# Autodesk Inventor assembly: GEYK1.0-70-10-B-10K
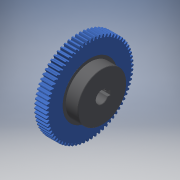
[picture p0: Inventor's stored thumbnail of the model, 180x180]
Saved by Autodesk Inventor 2019 (Build 230136000, 136)
## iProperties
Category: PARTsolutions
Company: MISUMI
Created: 2022-11-14
Part Number: GEYK1.0-70-10-B-10K
Catalog Web Link: www.cadenas.de
Description: GEY_-Plastic Bonded Spur Gears
Vendor: MISUMI
Document SubType Name: Assembly
Designer: psAdmin
Manufacturer: MISUMI
Mass: 49.0279 g
Surface Area: 167.17 cm^2
Volume: 49.0279 cm^3
Density: 1 g/cm^3
Title: GEYK1.0-70-10-B-10K
Author: Cadenas PARTsolutions
Comments: Plastic Bonded Spur Gears
PSOL_IDENT_0: {$CADENAS_DATA/23d-libs/misumi/metric/54_spur_gears/gey_asmtab.prj},217 {VTYP=3D},{STYP=ASSTAB},{NB=
PSOL_IDENT_1: GEYK1.0-70-10-B-10K},{LINA=GEYK1.0-70-10-B-10K},{NN=GEY_},{DATE=07.06.2021 01:25:59},{GEOMDATE=22.08
PSOL_IDENT_2: .2016 06:34:21},{VERSION=},{LINEID=10},{WBVAR=SHS,NT,PS,ALT1,ALT2,BS},{WBNUMERIC=NT,BS}  {NB=GEYK1.0
PSOL_IDENT_3: -70-10-B-10K},{LINA=GEYK1.0-70-10-B-10K},{KT=DUMMY},{PN=GEYK1.0-70-10-B-10K},{SHS=K},{SHSPN=K},{GEAK
PSOL_IDENT_4: BH=0},{MAT=MC Nylon},{MATC=S25C},{AC=Set Screw},{MOD=1.0},{NT=70},{NTA=30,32,34,35,36,38,40,42,45,48
PSOL_IDENT_5: ,50,52,56,60,70,75},{B=10},{TS=B},{TSA='B','B'},{PS=10K},{PSA= '10N','10N','10K','10K','11N','11N','
PSOL_IDENT_6: 12N','12N','13N','13N','14N','14N','15N','15N','16N','16N','17N','17N','18N','18N','19N','19N','20N'
PSOL_IDENT_7: ,'20N','21N','21N','22N','22N','23N','23N','24N','24N'},{PS1= '10','10','11','11','12','12','13','13'
PSOL_IDENT_8: ,'14','14','15','15','16','16','17','17','18','18','19','19','20','20','21','21','22','22','23','23'
PSOL_IDENT_9: ,'24','24','25','25','26','26','27','27','28','28'},{PS2= '10N','10N','10K','10K','11N','11N','12N','
PSOL_IDENT_10: 12N','13N','13N','14N','14N','15N','15N','16N','16N','17N','17N','18N','18N','19N','19N','20N','20N'
PSOL_IDENT_11: ,'21N','21N','22N','22N','23N','23N','24N','24N'},{P=10.00},{DD=70.0},{D=72.0},{H=40},{E=45},{L=20},
PSOL_IDENT_12: {LL=10},{LL2=5.000},{M=M4},{M2=4},{ACSS=M4x3},{TT=1.8},{BB=4},{ALT1=},{ALTA='','w/o Set Screw', '-KC
PSOL_IDENT_13: 90', 'with KC90 (Set Screw)', '-KC120', 'with KC120 (Set Screw)'},{SCREWL=3},{PLANE=20},{PLANE1=20},
PSOL_IDENT_14: {ALT2=},{ALT2A='','w/o Boss Cut','-BS','with BS (Boss Cut)'},{BS=0.0},{BSA=0},{BSMIN=7.0},{BSMAX=9.5
PSOL_IDENT_15: },{HD=15.000},{PPATH=gey_asmtpl.prj}
NB: GEYK1.0-70-10-B-10K
NN: GEY_
NT: 70
NBSYN: $PN.
LINA: GEYK1.0-70-10-B-10K
CATALOG: Misumi
PN: GEYK1.0-70-10-B-10K
SHS: Key Groove Hole+Tap
MAT: MC Nylon
MATC: S25C
AC: Set Screw
MOD: 1.0
B: 10
TS: B
PS: 10K
DD: 70
D: 72
H: 40
E: 45
L: 20
LL: 10
M: M4
ALT1: w/o Set Screw
ALT2: w/o Boss Cut
BS: 0
SUPPLIER: MISUMI
ARTICLENO: GEYK1.0-70-10-B-10K
BOMINFO: GEYK1.0-70-10-B-10K
CREATOR: CADENAS GmbH
## Documents named in this file (4)
- e:\temp\worker_COMMON_6\temp\tmp_4032_386_yddUP\format_0\GEYK1_0-70-10-B-10K.iam
- e:\temp\worker_COMMON_6\temp\tmp_4032_386_yddUP\format_0\GEYK1_0-70-10-B-10K_0_b.ipt
- e:\temp\worker_COMMON_6\temp\tmp_4032_386_yddUP\format_0\Hexagon socket set screw with flat point DIN 913 - M4x3.ipt
- e:\temp\worker_COMMON_6\temp\tmp_4032_386_yddUP\format_0\GEYK1_0-70-10-B-10K_0_t.ipt
## Components (3 placed, 3 different names)
1. GEYK1_0-70-10-B-10K_0_b:1 — screw1_XY@1 <-> IP1_XY@2, screw1_Z@1 <-> IP1_Z@2, screw1_YZ@1 <-> IP1_YZ@2, body_to_teeth_XY@1 <-> teeth_to_body_XY@3, body_to_teeth_Z@1 <-> teeth_to_body_Z@3, body_to_teeth_YZ@1 <-> teeth_to_body_YZ@3
2. Hexagon socket set screw with flat point DIN 913 - M4x3:1 — screw1_XY@1 <-> IP1_XY@2, screw1_Z@1 <-> IP1_Z@2, screw1_YZ@1 <-> IP1_YZ@2
3. GEYK1_0-70-10-B-10K_0_t:1 — body_to_teeth_XY@1 <-> teeth_to_body_XY@3, body_to_teeth_Z@1 <-> teeth_to_body_Z@3, body_to_teeth_YZ@1 <-> teeth_to_body_YZ@3
## Relationships (6: Mate 3, Angle 2, Flush 1)
- screw1_XY@1 <-> IP1_XY@2 [Flush]: GEYK1_0-70-10-B-10K_0_b:1 ↔ Hexagon socket set screw with flat point DIN 913 - M4x3:1
- screw1_Z@1 <-> IP1_Z@2 [Mate]: GEYK1_0-70-10-B-10K_0_b:1 ↔ Hexagon socket set screw with flat point DIN 913 - M4x3:1
- screw1_YZ@1 <-> IP1_YZ@2 [Angle] (0 deg): GEYK1_0-70-10-B-10K_0_b:1 ↔ Hexagon socket set screw with flat point DIN 913 - M4x3:1
- body_to_teeth_XY@1 <-> teeth_to_body_XY@3 [Mate]: GEYK1_0-70-10-B-10K_0_b:1 ↔ GEYK1_0-70-10-B-10K_0_t:1
- body_to_teeth_Z@1 <-> teeth_to_body_Z@3 [Mate]: GEYK1_0-70-10-B-10K_0_b:1 ↔ GEYK1_0-70-10-B-10K_0_t:1
- body_to_teeth_YZ@1 <-> teeth_to_body_YZ@3 [Angle] (0 deg): GEYK1_0-70-10-B-10K_0_b:1 ↔ GEYK1_0-70-10-B-10K_0_t:1
